# Autodesk Inventor assembly: AnsysModel
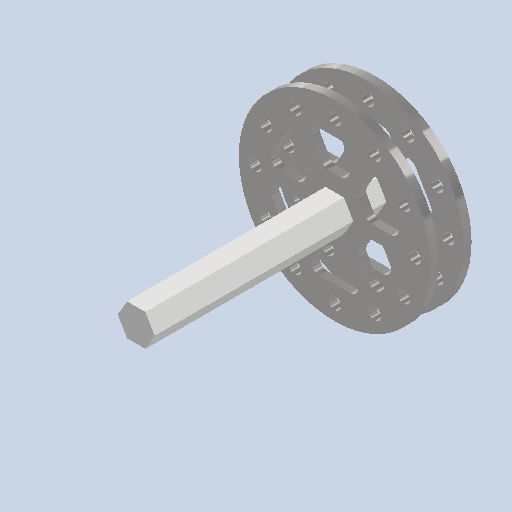
[picture p0: Inventor's stored thumbnail of the model, 512x512]
Saved by Autodesk Inventor 2025.1 (Build 291241020, 241B)
## iProperties
Created: 2023-05-01
Part Number: AnsysModel
Document SubType Name: Assembly
Designer: asach
Author: asach
## Documents named in this file (3)
- C:\Users\t205b\OneDrive\Documents\Github\BehrendURCMechanical\CAD\Chassis V3\Wheel\AnsysModel.iam
- C:\Users\t205b\OneDrive\Documents\Github\BehrendURCMechanical\CAD\Chassis V3\Wheel\AnsysHex.ipt
- C:\Users\t205b\OneDrive\Documents\Github\BehrendURCMechanical\CAD\Chassis V3\Wheel\ThickWheelPlate_v8.ipt
## Components (3 placed, 2 different names)
1. AnsysHex:1 — Mate:3, Mate:4, Flush:1
2. ThickWheelPlate_v8:1 — Mate:1, Mate:2, Mate:3, Mate:4, Mate:5
3. ThickWheelPlate_v8:2 — Mate:1, Mate:2, Mate:5, Flush:1
## Relationships (6: Mate 5, Flush 1)
- Mate:1: ThickWheelPlate_v8:1 ↔ ThickWheelPlate_v8:2
- Mate:2: ThickWheelPlate_v8:1 ↔ ThickWheelPlate_v8:2
- Mate:3: AnsysHex:1 ↔ ThickWheelPlate_v8:1
- Mate:4: AnsysHex:1 ↔ ThickWheelPlate_v8:1
- Mate:5 (10 mm): ThickWheelPlate_v8:1 ↔ ThickWheelPlate_v8:2
- Flush:1: AnsysHex:1 ↔ ThickWheelPlate_v8:2
